# Autodesk Inventor assembly: Inner shield New
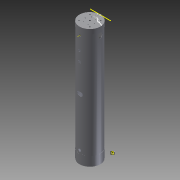
[picture p0: Inventor's stored thumbnail of the model, 180x180]
Saved by Autodesk Inventor 2015 (Build 190159000, 159)
## iProperties
Created: 2005-07-05
Part Number: Inner shield New
Document SubType Name: Assembly
Designer: jony
Author: jony
## Documents named in this file (4)
- C:\ColdMatter\CADFiles\EDM Machine\EDM Inner Shield\Inner Shield.iam
- C:\ColdMatter\CADFiles\EDM Machine\EDM Inner Shield\New Centre Section.ipt
- C:\ColdMatter\CADFiles\EDM Machine\EDM Inner Shield\bottom cap.ipt
- C:\ColdMatter\CADFiles\EDM Machine\EDM Inner Shield\top cap.ipt
## Components (3 placed, 3 different names)
1. New Centre Section:1 — Angle:1, Angle:2, Insert:1, Insert:2
2. bottom cap:1 — Angle:2, Insert:2
3. top cap:1 — Angle:1, Insert:1
## Relationships (4: Angle 2, Insert 2)
- Angle:1 (90 deg): New Centre Section:1 ↔ top cap:1
- Angle:2 (0 deg): New Centre Section:1 ↔ bottom cap:1
- Insert:1: New Centre Section:1 ↔ top cap:1
- Insert:2: New Centre Section:1 ↔ bottom cap:1
